# Autodesk Inventor assembly: recyclebine
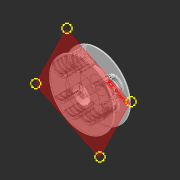
[picture p0: Inventor's stored thumbnail of the model, 180x180]
Saved by Autodesk Inventor 2020.3 (Build 243373010, 373A)
## iProperties
Created: 2021-02-15
Part Number: recyclebine
Document SubType Name: Assembly
Designer: Melvin Strobl
Author: Melvin Strobl
## Documents named in this file (3)
- X:\waterturbine\recyclebine\recyclebine.iam
- X:\waterturbine\recyclebine\spool.ipt
- X:\waterturbine\recyclebine\claw.ipt
## Components (8 placed, 2 different names)
1. spool:1 — Mate:2, Mate:10, Mate:11, Mate:12, Mate:14, Mate:15, Mate:16, Angle:1, Angle:2, Angle:4, Angle:5, Angle:6, Angle:8, Angle:9, Mate:18, Mate:19, Mate:21, Mate:22, Mate:23, Mate:24, Mate:25
2. claw:1 — Mate:2, Angle:4, Mate:24
3. claw:2 — Mate:10, Angle:8, Mate:25
4. claw:3 — Mate:11, Angle:2, Mate:18
5. claw:4 — Mate:12, Angle:1, Mate:19
6. claw:6 — Mate:14, Angle:6, Mate:21
7. claw:7 — Mate:15, Angle:9, Mate:22
8. claw:8 — Mate:16, Angle:5, Mate:23
## Relationships (21: Mate 14, Angle 7)
- Mate:2 (0.25 mm): spool:1 ↔ claw:1
- Mate:10 (0.25 mm): spool:1 ↔ claw:2
- Mate:11 (0.5 mm): spool:1 ↔ claw:3
- Mate:12 (0.25 mm): spool:1 ↔ claw:4
- Mate:14 (0.25 mm): spool:1 ↔ claw:6
- Mate:15 (0.25 mm): spool:1 ↔ claw:7
- Mate:16 (0.25 mm): spool:1 ↔ claw:8
- Angle:1 (0 deg): spool:1 ↔ claw:4
- Angle:2 (-65 deg): spool:1 ↔ claw:3
- Angle:4 (96 deg): spool:1 ↔ claw:1
- Angle:5 (98 deg): spool:1 ↔ claw:8
- Angle:6 (98 deg): spool:1 ↔ claw:6
- Angle:8 (-93 deg): spool:1 ↔ claw:2
- Angle:9 (-98 deg): spool:1 ↔ claw:7
- Mate:18: spool:1 ↔ claw:3
- Mate:19: spool:1 ↔ claw:4
- Mate:21: spool:1 ↔ claw:6
- Mate:22: spool:1 ↔ claw:7
- Mate:23: spool:1 ↔ claw:8
- Mate:24: spool:1 ↔ claw:1
- Mate:25: spool:1 ↔ claw:2
